# Autodesk Inventor assembly: Tank tread segment (Long) example.
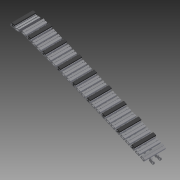
[picture p0: Inventor's stored thumbnail of the model, 180x180]
Saved by Autodesk Inventor 2015 (Build 190159000, 159)
## iProperties
Created: 2015-09-30
Part Number: Tank tread segment (Long) example.
Document SubType Name: Assembly
Designer: alhohbein
Author: alhohbein
## Documents named in this file (3)
- U:\Tank tread segment (Long) example..iam
- U:\TETRIX_736468_TT_LINK_2012.ipt
- U:\Tank tread with rubber insert.iam
## Components (27 placed, 2 different names)
1. TETRIX_736468_TT_LINK_2012:1 — Insert:1, Insert:30
2. TETRIX_736468_TT_LINK_2012:2 — Insert:1, Insert:2
3. Tank tread with rubber insert:1 [sub-assembly] — Insert:11, Insert:12
4. Tank tread with rubber insert:2 [sub-assembly] — Insert:5, Insert:6
5. Tank tread with rubber insert:3 [sub-assembly] — Insert:14, Insert:15
6. Tank tread with rubber insert:4 [sub-assembly] — Insert:8, Insert:9
7. Tank tread with rubber insert:5 [sub-assembly] — Insert:2, Insert:3
8. TETRIX_736468_TT_LINK_2012:3 — Insert:7, Insert:8
9. TETRIX_736468_TT_LINK_2012:4 — Insert:4, Insert:5
10. TETRIX_736468_TT_LINK_2012:5 — Insert:6, Insert:7
11. TETRIX_736468_TT_LINK_2012:6 — Insert:3, Insert:4
12. TETRIX_736468_TT_LINK_2012:7 — Insert:12, Insert:13
13. TETRIX_736468_TT_LINK_2012:8 — Insert:13, Insert:14
14. TETRIX_736468_TT_LINK_2012:9 — Insert:9, Insert:10
15. TETRIX_736468_TT_LINK_2012:10 — Insert:10, Insert:11
16. TETRIX_736468_TT_LINK_2012:11 — Insert:24, Insert:25
17. TETRIX_736468_TT_LINK_2012:12 — Insert:21, Insert:22
18. TETRIX_736468_TT_LINK_2012:13 — Insert:22, Insert:23
19. TETRIX_736468_TT_LINK_2012:14 — Insert:16, Insert:17
20. TETRIX_736468_TT_LINK_2012:15 — Insert:15, Insert:16
21. TETRIX_736468_TT_LINK_2012:16 — Insert:19, Insert:20
22. TETRIX_736468_TT_LINK_2012:18 — Insert:18, Insert:19
23. TETRIX_736468_TT_LINK_2012:20 — Insert:25
24. Tank tread with rubber insert:6 [sub-assembly] — Insert:17, Insert:18
25. Tank tread with rubber insert:7 [sub-assembly] — Insert:30
26. Tank tread with rubber insert:9 [sub-assembly] — Insert:20, Insert:21
27. Tank tread with rubber insert:10 [sub-assembly] — Insert:23, Insert:24
## Relationships (26: Insert 26)
- Insert:1: TETRIX_736468_TT_LINK_2012:1 ↔ TETRIX_736468_TT_LINK_2012:2
- Insert:2: TETRIX_736468_TT_LINK_2012:2 ↔ Tank tread with rubber insert:5
- Insert:3: Tank tread with rubber insert:5 ↔ TETRIX_736468_TT_LINK_2012:6
- Insert:4: TETRIX_736468_TT_LINK_2012:4 ↔ TETRIX_736468_TT_LINK_2012:6
- Insert:5: Tank tread with rubber insert:2 ↔ TETRIX_736468_TT_LINK_2012:4
- Insert:6: Tank tread with rubber insert:2 ↔ TETRIX_736468_TT_LINK_2012:5
- Insert:7: TETRIX_736468_TT_LINK_2012:3 ↔ TETRIX_736468_TT_LINK_2012:5
- Insert:8: Tank tread with rubber insert:4 ↔ TETRIX_736468_TT_LINK_2012:3
- Insert:9: Tank tread with rubber insert:4 ↔ TETRIX_736468_TT_LINK_2012:9
- Insert:10: TETRIX_736468_TT_LINK_2012:9 ↔ TETRIX_736468_TT_LINK_2012:10
- Insert:11: Tank tread with rubber insert:1 ↔ TETRIX_736468_TT_LINK_2012:10
- Insert:12: Tank tread with rubber insert:1 ↔ TETRIX_736468_TT_LINK_2012:7
- Insert:13: TETRIX_736468_TT_LINK_2012:7 ↔ TETRIX_736468_TT_LINK_2012:8
- Insert:14: Tank tread with rubber insert:3 ↔ TETRIX_736468_TT_LINK_2012:8
- Insert:15: Tank tread with rubber insert:3 ↔ TETRIX_736468_TT_LINK_2012:15
- Insert:16: TETRIX_736468_TT_LINK_2012:14 ↔ TETRIX_736468_TT_LINK_2012:15
- Insert:17: TETRIX_736468_TT_LINK_2012:14 ↔ Tank tread with rubber insert:6
- Insert:18: TETRIX_736468_TT_LINK_2012:18 ↔ Tank tread with rubber insert:6
- Insert:19: TETRIX_736468_TT_LINK_2012:16 ↔ TETRIX_736468_TT_LINK_2012:18
- Insert:20: TETRIX_736468_TT_LINK_2012:16 ↔ Tank tread with rubber insert:9
- Insert:21: TETRIX_736468_TT_LINK_2012:12 ↔ Tank tread with rubber insert:9
- Insert:22: TETRIX_736468_TT_LINK_2012:12 ↔ TETRIX_736468_TT_LINK_2012:13
- Insert:23: TETRIX_736468_TT_LINK_2012:13 ↔ Tank tread with rubber insert:10
- Insert:24: TETRIX_736468_TT_LINK_2012:11 ↔ Tank tread with rubber insert:10
- Insert:25: TETRIX_736468_TT_LINK_2012:11 ↔ TETRIX_736468_TT_LINK_2012:20
- Insert:30: TETRIX_736468_TT_LINK_2012:1 ↔ Tank tread with rubber insert:7
